# Autodesk Inventor assembly: Frame
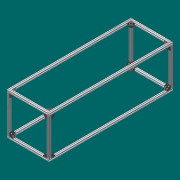
[picture p0: Inventor's stored thumbnail of the model, 180x180]
Saved by Autodesk Inventor 2016 SP1 (Build 200210100, 210)
## iProperties
Created: 2015-06-02
Part Number: Frame
Document SubType Name: Assembly
Designer: Sawaiz Syed
Author: Sawaiz Syed
## Documents named in this file (3)
- C:\Users\Sawaiz\OneDrive\projects\modularRICH\testMount\frame\frame.iam
- C:\Users\Sawaiz\OneDrive\projects\modularRICH\testMount\frame\frameHorizontal.iam
- C:\Users\Sawaiz\OneDrive\projects\modularRICH\testMount\frame\verticalStrut.iam
## Components (6 placed, 2 different names)
1. frameHorizontal:1 [sub-assembly] — Flush:1, Flush:2, Flush:3, Flush:4, Flush:7, Flush:8, Flush:12, Flush:13, Mate:1
2. frameHorizontal:2 [sub-assembly] — Flush:14, Flush:15, Mate:2
3. verticalStrut:1 [sub-assembly] — Flush:1, Flush:2, Flush:9, Flush:10
4. verticalStrut:2 [sub-assembly] — Flush:3, Flush:4, Flush:10, Flush:11
5. verticalStrut:3 [sub-assembly] — Flush:11, Flush:12, Flush:13, Mate:1
6. verticalStrut:4 [sub-assembly] — Flush:7, Flush:8, Flush:9, Flush:14, Flush:15, Mate:2
## Relationships (15: Flush 13, Mate 2)
- Flush:1: frameHorizontal:1 ↔ verticalStrut:1
- Flush:2: frameHorizontal:1 ↔ verticalStrut:1
- Flush:3: frameHorizontal:1 ↔ verticalStrut:2
- Flush:4: frameHorizontal:1 ↔ verticalStrut:2
- Flush:7: frameHorizontal:1 ↔ verticalStrut:4
- Flush:8: frameHorizontal:1 ↔ verticalStrut:4
- Flush:9: verticalStrut:1 ↔ verticalStrut:4
- Flush:10: verticalStrut:1 ↔ verticalStrut:2
- Flush:11: verticalStrut:2 ↔ verticalStrut:3
- Flush:12: frameHorizontal:1 ↔ verticalStrut:3
- Flush:13: frameHorizontal:1 ↔ verticalStrut:3
- Mate:1: frameHorizontal:1 ↔ verticalStrut:3
- Flush:14: frameHorizontal:2 ↔ verticalStrut:4
- Flush:15: frameHorizontal:2 ↔ verticalStrut:4
- Mate:2: frameHorizontal:2 ↔ verticalStrut:4
